# Autodesk Inventor assembly: testframe
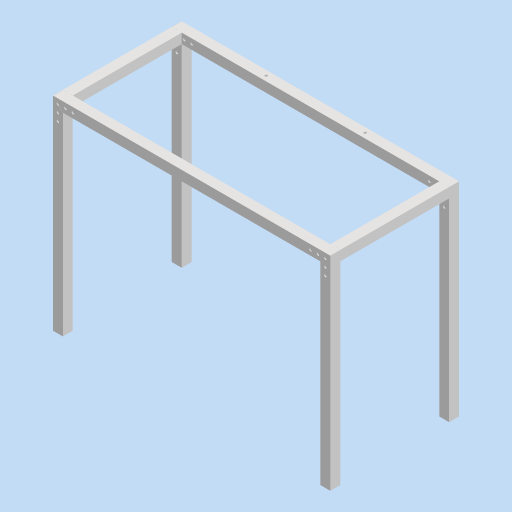
[picture p0: Inventor's stored thumbnail of the model, 512x512]
Saved by Autodesk Inventor 2024.3 (Build 283343000, 343)
## iProperties
Created: 2024-07-23
Part Number: testframe
Document SubType Name: Assembly
Designer: bryan
Author: bryan
## Documents named in this file (7)
- C:\Users\bryan\OneDrive\Documentos\GitHub\1622-2024-Summer-CAD-A-Thon\Structure\testframe.iam
- C:\Users\bryan\OneDrive\Documentos\GitHub\1622-2024-Summer-CAD-A-Thon\Structure\STRU_001_BilletBlock.ipt
- C:\Users\bryan\OneDrive\Documentos\GitHub\1622-2024-Summer-CAD-A-Thon\Structure\STRU_002_BilletPole_20.56in_Angled.ipt
- C:\Users\bryan\OneDrive\Documentos\GitHub\1622-2024-Summer-CAD-A-Thon\Structure\STRU_003_BilletPole_28in_Angled.ipt
- C:\Users\bryan\OneDrive\Documentos\GitHub\1622-2024-Summer-CAD-A-Thon\Structure\STRU_004_DoubleBillet_90_2.25in.ipt
- C:\Users\bryan\OneDrive\Documentos\GitHub\1622-2024-Summer-CAD-A-Thon\Structure\STRU_006_BilletPole_11in.ipt
- C:\Users\bryan\OneDrive\Documentos\GitHub\1622-2024-Summer-CAD-A-Thon\Structure\STRU_003_BilletPole_28in_Angled_Unique.ipt
## Components (20 placed, 6 different names)
1. STRU_001_BilletBlock:2 — Mate:16, Mate:17, Flush:2
2. STRU_002_BilletPole_20.56in_Angled:1 — Mate:1, Mate:4, Mate:5, Flush:5, Mate:41, Mate:53, Mate:54, Flush:10
3. STRU_004_DoubleBillet_90_2.25in:1 — Mate:1, Mate:4, Mate:5, Mate:34, Mate:56, Mate:58
4. STRU_002_BilletPole_20.56in_Angled:2 — Mate:13, Mate:14, Mate:15, Mate:16, Mate:17, Flush:2, Mate:40
5. STRU_004_DoubleBillet_90_2.25in:2 — Mate:13, Mate:14, Mate:15, Mate:36, Mate:57
6. STRU_001_BilletBlock:3
7. STRU_001_BilletBlock:4
8. STRU_002_BilletPole_20.56in_Angled:3 — Flush:5, Mate:39
9. STRU_003_BilletPole_28in_Angled:2 — Mate:47, Flush:8, Flush:9, Mate:55
10. STRU_004_DoubleBillet_90_2.25in:3 — Mate:35
11. STRU_002_BilletPole_20.56in_Angled:4 — Mate:38
12. STRU_004_DoubleBillet_90_2.25in:4 — Mate:37
13. STRU_001_BilletBlock:5 — Mate:34, Mate:41, Mate:50, Mate:51
14. STRU_001_BilletBlock:6 — Mate:35, Mate:39, Mate:48, Mate:49
15. STRU_001_BilletBlock:7 — Mate:37, Mate:38, Mate:45, Mate:46
16. STRU_001_BilletBlock:8 — Mate:36, Mate:40, Mate:42, Mate:43
17. STRU_006_BilletPole_11in:1 — Mate:48, Mate:49, Flush:9, Mate:50, Mate:51, Mate:55, Mate:59
18. STRU_006_BilletPole_11in:2 — Mate:42, Mate:43, Mate:45, Mate:46, Mate:47, Flush:8
19. STRU_001_BilletBlock:9 — Mate:53, Mate:54, Flush:10
20. STRU_003_BilletPole_28in_Angled_Unique:1 — Mate:56, Mate:57, Mate:58, Mate:59
## Relationships (55: Mate 48, Flush 7)
- Mate:1: STRU_002_BilletPole_20.56in_Angled:1 ↔ STRU_004_DoubleBillet_90_2.25in:1
- Mate:4: STRU_002_BilletPole_20.56in_Angled:1 ↔ STRU_004_DoubleBillet_90_2.25in:1
- Mate:5: STRU_002_BilletPole_20.56in_Angled:1 ↔ STRU_004_DoubleBillet_90_2.25in:1
- Mate:13: STRU_002_BilletPole_20.56in_Angled:2 ↔ STRU_004_DoubleBillet_90_2.25in:2
- Mate:14: STRU_002_BilletPole_20.56in_Angled:2 ↔ STRU_004_DoubleBillet_90_2.25in:2
- Mate:15: STRU_002_BilletPole_20.56in_Angled:2 ↔ STRU_004_DoubleBillet_90_2.25in:2
- Mate:16: STRU_001_BilletBlock:2 ↔ STRU_002_BilletPole_20.56in_Angled:2
- Mate:17: STRU_001_BilletBlock:2 ↔ STRU_002_BilletPole_20.56in_Angled:2
- Flush:2: STRU_001_BilletBlock:2 ↔ STRU_002_BilletPole_20.56in_Angled:2
- [Mate]: STRU_002_BilletPole_20.56in_Angled:3 ↔ STRU_004_DoubleBillet_90_2.25in:3
- [Mate]: STRU_001_BilletBlock:3 ↔ STRU_002_BilletPole_20.56in_Angled:3
- [Mate]: STRU_001_BilletBlock:3 ↔ STRU_002_BilletPole_20.56in_Angled:3
- [Flush]: STRU_001_BilletBlock:3 ↔ STRU_002_BilletPole_20.56in_Angled:3
- [Mate]: STRU_002_BilletPole_20.56in_Angled:3 ↔ STRU_004_DoubleBillet_90_2.25in:3
- [Mate]: STRU_002_BilletPole_20.56in_Angled:3 ↔ STRU_004_DoubleBillet_90_2.25in:3
- [Mate]: STRU_003_BilletPole_28in_Angled:2 ↔ STRU_004_DoubleBillet_90_2.25in:3
- [Mate]: STRU_003_BilletPole_28in_Angled:2 ↔ STRU_004_DoubleBillet_90_2.25in:3
- [Mate]: STRU_003_BilletPole_28in_Angled:2 ↔ STRU_004_DoubleBillet_90_2.25in:3
- [Mate]: STRU_003_BilletPole_28in_Angled:2 ↔ STRU_004_DoubleBillet_90_2.25in:4
- [Mate]: STRU_003_BilletPole_28in_Angled:2 ↔ STRU_004_DoubleBillet_90_2.25in:4
- [Mate]: STRU_003_BilletPole_28in_Angled:2 ↔ STRU_004_DoubleBillet_90_2.25in:4
- [Mate]: STRU_002_BilletPole_20.56in_Angled:4 ↔ STRU_004_DoubleBillet_90_2.25in:4
- [Mate]: STRU_002_BilletPole_20.56in_Angled:4 ↔ STRU_004_DoubleBillet_90_2.25in:4
- [Mate]: STRU_002_BilletPole_20.56in_Angled:4 ↔ STRU_004_DoubleBillet_90_2.25in:4
- [Mate]: STRU_001_BilletBlock:4 ↔ STRU_002_BilletPole_20.56in_Angled:4
- [Mate]: STRU_001_BilletBlock:4 ↔ STRU_002_BilletPole_20.56in_Angled:4
- [Flush]: STRU_001_BilletBlock:4 ↔ STRU_002_BilletPole_20.56in_Angled:4
- Flush:5: STRU_002_BilletPole_20.56in_Angled:1 ↔ STRU_002_BilletPole_20.56in_Angled:3
- Mate:34: STRU_004_DoubleBillet_90_2.25in:1 ↔ STRU_001_BilletBlock:5
- Mate:35: STRU_004_DoubleBillet_90_2.25in:3 ↔ STRU_001_BilletBlock:6
- Mate:36: STRU_004_DoubleBillet_90_2.25in:2 ↔ STRU_001_BilletBlock:8
- Mate:37: STRU_004_DoubleBillet_90_2.25in:4 ↔ STRU_001_BilletBlock:7
- Mate:38: STRU_002_BilletPole_20.56in_Angled:4 ↔ STRU_001_BilletBlock:7
- Mate:39: STRU_002_BilletPole_20.56in_Angled:3 ↔ STRU_001_BilletBlock:6
- Mate:40: STRU_002_BilletPole_20.56in_Angled:2 ↔ STRU_001_BilletBlock:8
- Mate:41: STRU_002_BilletPole_20.56in_Angled:1 ↔ STRU_001_BilletBlock:5
- Mate:42: STRU_001_BilletBlock:8 ↔ STRU_006_BilletPole_11in:2
- Mate:43: STRU_001_BilletBlock:8 ↔ STRU_006_BilletPole_11in:2
- Mate:45: STRU_001_BilletBlock:7 ↔ STRU_006_BilletPole_11in:2
- Mate:46: STRU_001_BilletBlock:7 ↔ STRU_006_BilletPole_11in:2
- Mate:47: STRU_003_BilletPole_28in_Angled:2 ↔ STRU_006_BilletPole_11in:2
- Flush:8: STRU_003_BilletPole_28in_Angled:2 ↔ STRU_006_BilletPole_11in:2
- Mate:48: STRU_001_BilletBlock:6 ↔ STRU_006_BilletPole_11in:1
- Mate:49: STRU_001_BilletBlock:6 ↔ STRU_006_BilletPole_11in:1
- Flush:9: STRU_003_BilletPole_28in_Angled:2 ↔ STRU_006_BilletPole_11in:1
- Mate:50: STRU_001_BilletBlock:5 ↔ STRU_006_BilletPole_11in:1
- Mate:51: STRU_001_BilletBlock:5 ↔ STRU_006_BilletPole_11in:1
- Mate:53: STRU_002_BilletPole_20.56in_Angled:1 ↔ STRU_001_BilletBlock:9
- Mate:54: STRU_002_BilletPole_20.56in_Angled:1 ↔ STRU_001_BilletBlock:9
- Flush:10: STRU_002_BilletPole_20.56in_Angled:1 ↔ STRU_001_BilletBlock:9
- Mate:55: STRU_003_BilletPole_28in_Angled:2 ↔ STRU_006_BilletPole_11in:1
- Mate:56: STRU_004_DoubleBillet_90_2.25in:1 ↔ STRU_003_BilletPole_28in_Angled_Unique:1
- Mate:57: STRU_004_DoubleBillet_90_2.25in:2 ↔ STRU_003_BilletPole_28in_Angled_Unique:1
- Mate:58: STRU_004_DoubleBillet_90_2.25in:1 ↔ STRU_003_BilletPole_28in_Angled_Unique:1
- Mate:59: STRU_006_BilletPole_11in:1 ↔ STRU_003_BilletPole_28in_Angled_Unique:1
## Named parameters: d19_d3 = 0 mm, d20_d4 = 0 mm, d21_d5 = 0 mm, d22_d7 = 0 mm, d23_d8 = 0 mm, d24_d9 = 0 mm, d25_d10 = 0 mm, d26_d11 = 0 mm, d27_d12 = 0 mm, d28_d13 = 0 mm, d29_d14 = 0 mm, d30_d15 = 0 mm, d31_d16 = 0 mm, d32_d17 = 0 mm, d33_d18 = 0 mm, d34_d0 = 0 mm, d35_d1 = 0 mm, d36_d2 = 0 mm
